# Autodesk Inventor assembly: toss up A bot gearbox
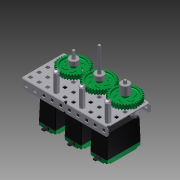
[picture p0: Inventor's stored thumbnail of the model, 180x180]
Saved by Autodesk Inventor 2014 SP1 (Build 180222100, 222)
## iProperties
Created: 2013-08-29
Part Number: toss up A bot gearbox
Document SubType Name: Assembly
Designer: Ryan
Sending System: SolidWorks 2013
Last Author: Ryan
Author: Ryan
## Documents named in this file (10)
- C:\Users\Ryan\Desktop\pack and go\Workspaces\Workspace\toss up 1st A bot\inventor drive\toss up A bot gearbox_MIR.iam
- C:\Users\Ryan\Desktop\pack and go\Workspaces\Workspace\lib\Aperture VEX CAD Library\Metal\C Channel\5 x 10.ipt
- C:\Users\Ryan\Desktop\pack and go\Workspaces\Workspace\toss up 1st A bot\inventor drive\toss up A bot one motor on gearbox.iam
- C:\Users\Ryan\Desktop\pack and go\Workspaces\Workspace\lib\Aperture VEX CAD Library\Shaft\2 inch Shaft.ipt
- C:\Users\Ryan\Desktop\pack and go\Workspaces\Workspace\lib\Aperture VEX CAD Library\Shaft\3 inch shaft.ipt
- C:\Users\Ryan\Desktop\pack and go\Workspaces\Workspace\lib\Super Sonic Sparks VEX CAD Library\Gears & Pulleys\36-Tooth Gear.ipt
- C:\Users\Ryan\Desktop\pack and go\Workspaces\Workspace\lib\Aperture VEX CAD Library\Standoffs\BEAM-1000.ipt
- C:\Users\Ryan\Desktop\pack and go\Workspaces\Workspace\lib\Aperture VEX CAD Library\Hardware\8-32\8-32_.375.ipt
- C:\Users\Ryan\Desktop\pack and go\Workspaces\Workspace\lib\Aperture VEX CAD Library\Spacers\spacer-0500-0250.ipt
- C:\Users\Ryan\Desktop\pack and go\Workspaces\Workspace\lib\Aperture VEX CAD Library\Spacers\spacer-0500-0500.ipt
## Components (22 placed, 10 different names)
1. 5 x 10:1 — Mate:21, Mate:22, Mate:23, Mate:24, Mate:33, Mate:34, Mate:35, Mate:37
2. 2 inch shaft:2 — Mate:11, Mate:12, Mate:26
3. 3 inch shaft:1 — Mate:17, Mate:18, Mate:29
4. 36-Tooth Gear:1 — Mate:5, Mate:11, Mate:12, Mate:25, Mate:40, Mate:41
5. 36-Tooth Gear:2 — Mate:14, Mate:15, Mate:30, Mate:31, Mate:44, Mate:45
6. 36-Tooth Gear:3 — Mate:17, Mate:18, Mate:27, Mate:28, Mate:42, Mate:43
7. 2 inch Shaft:3 — Mate:14, Mate:15, Mate:32
8. spacer-0500-0250:1 — Mate:40, Mate:41
9. spacer-0500-0250:2 — Mate:42, Mate:43
10. SPACER-0500-0500:1 — Mate:44, Mate:45
11. toss up A bot one motor on gearbox:3 [sub-assembly] — Mate:5, Mate:21, Mate:22, Mate:23, Mate:24, Mate:25, Mate:26
12. toss up A bot one motor on gearbox:4 [sub-assembly] — Mate:27, Mate:28, Mate:29
13. toss up A bot one motor on gearbox:5 [sub-assembly] — Mate:30, Mate:31, Mate:32
14. BEAM-1000:1 — Mate:33, Mate:34, Mate:35, Mate:36, Mate:38, Mate:39
15. 8-32_.375:1 — Mate:36, Mate:37
16. 8-32_.375:4 — Mate:38, Mate:39
17. BEAM-1000:2
18. 8-32_.375:2
19. 8-32_.375:5
20. BEAM-1000:3
21. 8-32_.375:3
22. 8-32_.375:6
## Component patterns: (3 elements, first: toss up A bot one motor on gearbox:3), (3 elements, first: BEAM-1000:1 + 8-32_.375:1 + 8-32_.375:4)
## Relationships (32: Mate 32)
- Mate:5: 36-Tooth Gear:1 ↔ toss up A bot one motor on gearbox:3
- Mate:11 (0.025 mm): 2 inch shaft:2 ↔ 36-Tooth Gear:1
- Mate:12 (0.025 mm): 2 inch shaft:2 ↔ 36-Tooth Gear:1
- Mate:14 (0.025 mm): 36-Tooth Gear:2 ↔ 2 inch Shaft:3
- Mate:15 (0.025 mm): 36-Tooth Gear:2 ↔ 2 inch Shaft:3
- Mate:17 (0.025 mm): 3 inch shaft:1 ↔ 36-Tooth Gear:3
- Mate:18 (0.025 mm): 3 inch shaft:1 ↔ 36-Tooth Gear:3
- Mate:21: 5 x 10:1 ↔ toss up A bot one motor on gearbox:3
- Mate:22 (-10.3886 mm): 5 x 10:1 ↔ toss up A bot one motor on gearbox:3
- Mate:23 (2.3114 mm): 5 x 10:1 ↔ toss up A bot one motor on gearbox:3
- Mate:24 (15.0114 mm): 5 x 10:1 ↔ toss up A bot one motor on gearbox:3
- Mate:25: 36-Tooth Gear:1 ↔ toss up A bot one motor on gearbox:3
- Mate:26: 2 inch shaft:2 ↔ toss up A bot one motor on gearbox:3
- Mate:27: 36-Tooth Gear:3 ↔ toss up A bot one motor on gearbox:4
- Mate:28: 36-Tooth Gear:3 ↔ toss up A bot one motor on gearbox:4
- Mate:29: 3 inch shaft:1 ↔ toss up A bot one motor on gearbox:4
- Mate:30: 36-Tooth Gear:2 ↔ toss up A bot one motor on gearbox:5
- Mate:31: 36-Tooth Gear:2 ↔ toss up A bot one motor on gearbox:5
- Mate:32: 2 inch Shaft:3 ↔ toss up A bot one motor on gearbox:5
- Mate:33: 5 x 10:1 ↔ BEAM-1000:1
- Mate:34 (2.3114 mm): 5 x 10:1 ↔ BEAM-1000:1
- Mate:35 (40.4114 mm): 5 x 10:1 ↔ BEAM-1000:1
- Mate:36: BEAM-1000:1 ↔ 8-32_.375:1
- Mate:37: 5 x 10:1 ↔ 8-32_.375:1
- Mate:38: BEAM-1000:1 ↔ 8-32_.375:4
- Mate:39 (1.1684 mm): BEAM-1000:1 ↔ 8-32_.375:4
- Mate:40: 36-Tooth Gear:1 ↔ spacer-0500-0250:1
- Mate:41: 36-Tooth Gear:1 ↔ spacer-0500-0250:1
- Mate:42: 36-Tooth Gear:3 ↔ spacer-0500-0250:2
- Mate:43: 36-Tooth Gear:3 ↔ spacer-0500-0250:2
- Mate:44: 36-Tooth Gear:2 ↔ SPACER-0500-0500:1
- Mate:45: 36-Tooth Gear:2 ↔ SPACER-0500-0500:1
## Named parameters: q = 2.3114 mm, sh = 0.025 mm, metal = 1.1684 mm
